# Autodesk Inventor assembly: motor assembly
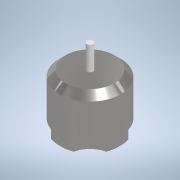
[picture p0: Inventor's stored thumbnail of the model, 180x180]
Saved by Autodesk Inventor 2021 (Build 250183000, 183)
## iProperties
Created: 2022-03-18
Part Number: motor assembly
Document SubType Name: Assembly
Designer: bobmu
Author: bobmu
## Documents named in this file (3)
- C:\Users\bobmu\Desktop\motor assembly.iam
- C:\Users\bobmu\Desktop\Part3.ipt
- C:\Users\bobmu\Desktop\Motor.ipt
## Components (2 placed, 2 different names)
1. Part3:1 — Insert:1
2. Motor:1 — Insert:1
## Relationships (1: Insert 1)
- Insert:1 (-11 mm): Part3:1 ↔ Motor:1
